# Autodesk Inventor assembly: Tray_Dropper_Asm
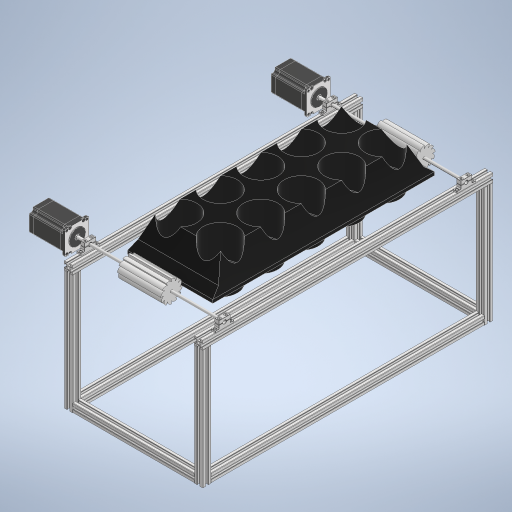
[picture p0: Inventor's stored thumbnail of the model, 512x512]
Saved by Autodesk Inventor 2023 (Build 270158000, 158)
## iProperties
Created: 2023-04-05
Part Number: Tray_Dropper_Asm
Document SubType Name: Assembly
Designer: Steven
_SolveAssemblyDoc: Frame Generator Solve Assembly
_Version: 25.0.0
Author: Steven
## Documents named in this file (7)
- C:\Users\steve\OneDrive\Documents\McMaster University\Courses-Year5\4TB6 Capstone Design Project\The_Nursery_Project\parts\Tray Dropper\ALTERNATIVE SOLUTION\Tray_Dropper_Asm.iam
- C:\Users\steve\OneDrive\Documents\McMaster University\Courses-Year5\4TB6 Capstone Design Project\The_Nursery_Project\parts\Tray Dropper\ALTERNATIVE SOLUTION\tray_dropper_frame_skeleton.ipt
- C:\Users\steve\OneDrive\Documents\McMaster University\Courses-Year5\4TB6 Capstone Design Project\The_Nursery_Project\parts\Tray Dropper\ALTERNATIVE SOLUTION\Tray_Dropper_Asm\Frame\Frame 1680721558395.iam
- C:\Users\steve\OneDrive\Documents\McMaster University\Courses-Year5\4TB6 Capstone Design Project\The_Nursery_Project\parts\Tray Dropper\ALTERNATIVE SOLUTION\WHEEL X SHAFT.iam
- C:\Users\steve\OneDrive\Documents\McMaster University\Courses-Year5\4TB6 Capstone Design Project\The_Nursery_Project\parts\Tray Dropper\Gantry\1865K21_Easy-Access Base-Mounted Shaft Support.ipt
- C:\Users\steve\OneDrive\Documents\McMaster University\Courses-Year5\4TB6 Capstone Design Project\The_Nursery_Project\parts\Tray Elevator\tray.ipt
- C:\Users\steve\OneDrive\Documents\McMaster University\Courses-Year5\4TB6 Capstone Design Project\The_Nursery_Project\parts\Tray Elevator\NEMA Stepper Motor.iam
## Components (11 placed, 6 different names)
1. tray_dropper_frame_skeleton:1
2. Frame 1680721558395:1 [sub-assembly] — Flush:2, Mate:2, Flush:3, Mate:3, Flush:4, Mate:4, Flush:5, Mate:5, Flush:7
3. WHEEL X SHAFT:1 [sub-assembly] — Mate:8, Mate:10, Mate:14, Mate:17
4. WHEEL X SHAFT:2 [sub-assembly] — Mate:11, Mate:12, Mate:13, Flush:6, Mate:19
5. 1865K21_Easy-Access Base-Mounted Shaft Support:1 — Flush:2, Mate:2, Mate:7, Mate:8, Mate:10, Mate:15, Angle:1, Mate:18
6. 1865K21_Easy-Access Base-Mounted Shaft Support:2 — Flush:3, Mate:3, Mate:6, Mate:11, Mate:12, Mate:15, Flush:7, Mate:16, Angle:2, Mate:20
7. 1865K21_Easy-Access Base-Mounted Shaft Support:3 — Flush:5, Mate:5, Mate:6
8. 1865K21_Easy-Access Base-Mounted Shaft Support:4 — Flush:4, Mate:4, Mate:7
9. tray:1 — Mate:13, Flush:6, Mate:14, Mate:16
10. NEMA Stepper Motor:1 [sub-assembly] — Mate:17, Angle:1, Mate:18
11. NEMA Stepper Motor:2 [sub-assembly] — Mate:19, Angle:2, Mate:20
## Relationships (26: Mate 18, Flush 6, Angle 2)
- Flush:2: Frame 1680721558395:1 ↔ 1865K21_Easy-Access Base-Mounted Shaft Support:1
- Mate:2: Frame 1680721558395:1 ↔ 1865K21_Easy-Access Base-Mounted Shaft Support:1
- Flush:3: Frame 1680721558395:1 ↔ 1865K21_Easy-Access Base-Mounted Shaft Support:2
- Mate:3: Frame 1680721558395:1 ↔ 1865K21_Easy-Access Base-Mounted Shaft Support:2
- Flush:4: Frame 1680721558395:1 ↔ 1865K21_Easy-Access Base-Mounted Shaft Support:4
- Mate:4: Frame 1680721558395:1 ↔ 1865K21_Easy-Access Base-Mounted Shaft Support:4
- Flush:5: Frame 1680721558395:1 ↔ 1865K21_Easy-Access Base-Mounted Shaft Support:3
- Mate:5: Frame 1680721558395:1 ↔ 1865K21_Easy-Access Base-Mounted Shaft Support:3
- Mate:6: 1865K21_Easy-Access Base-Mounted Shaft Support:2 ↔ 1865K21_Easy-Access Base-Mounted Shaft Support:3
- Mate:7: 1865K21_Easy-Access Base-Mounted Shaft Support:1 ↔ 1865K21_Easy-Access Base-Mounted Shaft Support:4
- Mate:8: WHEEL X SHAFT:1 ↔ 1865K21_Easy-Access Base-Mounted Shaft Support:1
- Mate:10: WHEEL X SHAFT:1 ↔ 1865K21_Easy-Access Base-Mounted Shaft Support:1
- Mate:11: WHEEL X SHAFT:2 ↔ 1865K21_Easy-Access Base-Mounted Shaft Support:2
- Mate:12: WHEEL X SHAFT:2 ↔ 1865K21_Easy-Access Base-Mounted Shaft Support:2
- Mate:13: WHEEL X SHAFT:2 ↔ tray:1
- Flush:6 (-50.8 mm): WHEEL X SHAFT:2 ↔ tray:1
- Mate:14: WHEEL X SHAFT:1 ↔ tray:1
- Mate:15 (523 mm): 1865K21_Easy-Access Base-Mounted Shaft Support:1 ↔ 1865K21_Easy-Access Base-Mounted Shaft Support:2
- Flush:7 (40 mm): Frame 1680721558395:1 ↔ 1865K21_Easy-Access Base-Mounted Shaft Support:2
- Mate:16 (1.5 mm): 1865K21_Easy-Access Base-Mounted Shaft Support:2 ↔ tray:1
- Mate:17: WHEEL X SHAFT:1 ↔ NEMA Stepper Motor:1
- Angle:1 (0 deg): 1865K21_Easy-Access Base-Mounted Shaft Support:1 ↔ NEMA Stepper Motor:1
- Mate:18: 1865K21_Easy-Access Base-Mounted Shaft Support:1 ↔ NEMA Stepper Motor:1
- Mate:19: WHEEL X SHAFT:2 ↔ NEMA Stepper Motor:2
- Angle:2 (0 deg): 1865K21_Easy-Access Base-Mounted Shaft Support:2 ↔ NEMA Stepper Motor:2
- Mate:20: 1865K21_Easy-Access Base-Mounted Shaft Support:2 ↔ NEMA Stepper Motor:2
